# Autodesk Inventor assembly: ведро с круто
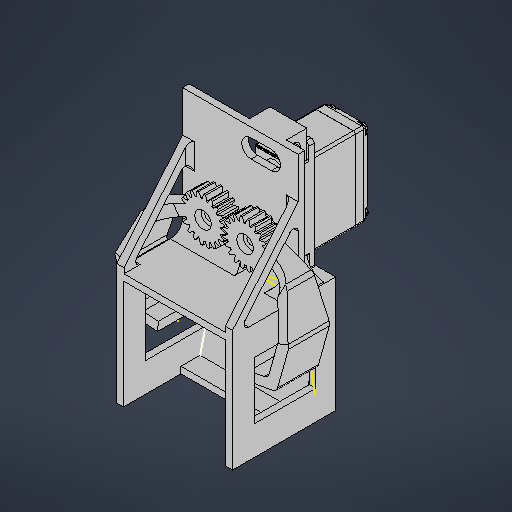
[picture p0: Inventor's stored thumbnail of the model, 512x512]
Saved by Autodesk Inventor 2025 (Build 290162000, 162)
## iProperties
Created: 2025-01-15
Part Number: ведро с круто
Document SubType Name: Assembly
Designer: Phantom
Author: Phantom
## Documents named in this file (6)
- C:\Users\Phantom\Desktop\Phantom16950\ведро с круто.iam
- C:\Users\Phantom\Desktop\Phantom16950\ведро.ipt
- C:\Users\Phantom\Desktop\Phantom16950\манипулятор 1.ipt
- C:\Users\Phantom\Downloads\am-5401 Sample\am-5401 Sample.ipt
- C:\Users\Phantom\Desktop\Phantom16950\манипулятор 1_MIR1.ipt
- C:\Users\Phantom\Desktop\Phantom16950\2000-0025-0002\2000-0025-0002.ipt
## Components (5 placed, 5 different names)
1. ведро:1 — Совмещение:1, Совмещение:3, Совмещение:5, Совмещение:6, Совмещение:10
2. am-5401 Sample:1 — Совмещение:1
3. манипулятор 1:1 — Совмещение:3
4. манипулятор 1_MIR1:1 — Совмещение:5, Совмещение:9
5. 2000-0025-0002:1 — Совмещение:6, Совмещение:9, Совмещение:10
## Relationships (6: Mate 6)
- Совмещение:1 [Mate]: ведро:1 ↔ am-5401 Sample:1
- Совмещение:3 [Mate]: ведро:1 ↔ манипулятор 1:1
- Совмещение:5 [Mate]: ведро:1 ↔ манипулятор 1_MIR1:1
- Совмещение:6 [Mate]: ведро:1 ↔ 2000-0025-0002:1
- Совмещение:9 [Mate]: манипулятор 1_MIR1:1 ↔ 2000-0025-0002:1
- Совмещение:10 [Mate]: ведро:1 ↔ 2000-0025-0002:1
